# Autodesk Inventor assembly: flat 0.125B
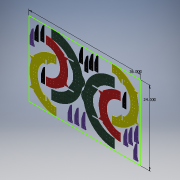
[picture p0: Inventor's stored thumbnail of the model, 180x180]
Saved by Autodesk Inventor 2016 (Build 200138000, 138)
## iProperties
Created: 2016-02-06
Part Number: flat 0.125B
Document SubType Name: Assembly
Designer: Scott
Author: Scott
## Documents named in this file (6)
- F:\Dropbox\CubeSat\Cleaned_Up_Helmholtz_Model_for_Manual\Flat_Patterns\flat 0.125B.iam
- F:\Dropbox\CubeSat\Cleaned_Up_Helmholtz_Model_for_Manual\Parts\Small_Coil_Outer.ipt
- F:\Dropbox\CubeSat\Cleaned_Up_Helmholtz_Model_for_Manual\Parts\Medium_Coil_Outer.ipt
- F:\Dropbox\CubeSat\Cleaned_Up_Helmholtz_Model_for_Manual\Parts\Large_Coil_Outer_Top.ipt
- F:\Dropbox\CubeSat\Cleaned_Up_Helmholtz_Model_for_Manual\Parts\Coil_Retainer_2_Hole.ipt
- F:\Dropbox\CubeSat\Cleaned_Up_Helmholtz_Model_for_Manual\Parts\Coil_Retainer_3_Hole.ipt
## Components (22 placed, 5 different names)
1. Large_Coil_Outer_Top:1
2. Large_Coil_Outer_Top:2
3. Medium_Coil_Outer:2 — Flush:8
4. Medium_Coil_Outer:1 — Flush:8
5. Small_Coil_Outer:2
6. Small_Coil_Outer:3
7. Coil_Retainer_2_Hole:1 — Flush:14
8. Coil_Retainer_2_Hole:2 — Flush:14
9. Coil_Retainer_2_Hole:3 — Flush:15, Flush:16
10. Coil_Retainer_2_Hole:4 — Flush:15
11. Coil_Retainer_2_Hole:5 — Flush:16, Flush:17
12. Coil_Retainer_2_Hole:6 — Flush:19
13. Coil_Retainer_2_Hole:7 — Flush:17, Flush:18
14. Coil_Retainer_2_Hole:8 — Flush:18, Flush:19
15. Coil_Retainer_3_Hole:1
16. Coil_Retainer_3_Hole:2
17. Coil_Retainer_3_Hole:3
18. Coil_Retainer_3_Hole:4
19. Coil_Retainer_3_Hole:5
20. Coil_Retainer_3_Hole:6
21. Coil_Retainer_3_Hole:7
22. Coil_Retainer_3_Hole:8
## Relationships (7: Flush 7)
- Flush:8: Medium_Coil_Outer:2 ↔ Medium_Coil_Outer:1
- Flush:14: Coil_Retainer_2_Hole:1 ↔ Coil_Retainer_2_Hole:2
- Flush:15: Coil_Retainer_2_Hole:3 ↔ Coil_Retainer_2_Hole:4
- Flush:16: Coil_Retainer_2_Hole:3 ↔ Coil_Retainer_2_Hole:5
- Flush:17: Coil_Retainer_2_Hole:5 ↔ Coil_Retainer_2_Hole:7
- Flush:18: Coil_Retainer_2_Hole:7 ↔ Coil_Retainer_2_Hole:8
- Flush:19: Coil_Retainer_2_Hole:6 ↔ Coil_Retainer_2_Hole:8
